# Autodesk Inventor assembly: HalfElevatpr
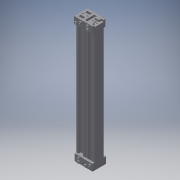
[picture p0: Inventor's stored thumbnail of the model, 180x180]
Saved by Autodesk Inventor 2019 (Build 230136000, 136)
## iProperties
Created: 2019-09-28
Part Number: HalfElevatpr
Document SubType Name: Assembly
Designer: james
Author: james
## Documents named in this file (5)
- F:\JimsDesign\Jims2020FTC\HalfElevatpr.iam
- F:\JimsDesign\Jims2020FTC\LeftSideElevator.ipt
- F:\JimsDesign\Library\McMaster\SocketScrews\91251A197_BLACK-OXIDE ALLOY STEEL SOCKET HEAD CAP SCREW.ipt
- F:\JimsDesign\Jims2020FTC\SliderLeft.iam
- F:\JimsDesign\Jims2020FTC\SliderRight.iam
## Components (8 placed, 4 different names)
1. LeftSideElevator:1 — Mate:8, Mate:9, Mate:14, Mate:15, Flush:2
2. LeftSideElevator:2 — Mate:16, Mate:17, Mate:18, Mate:19, Flush:3, Mate:20, Mate:21, Flush:4
3. 91251A197_BLACK-OXIDE ALLOY STEEL SOCKET HEAD CAP SCREW:1 — Mate:12, Mate:13
4. 91251A197_BLACK-OXIDE ALLOY STEEL SOCKET HEAD CAP SCREW:2 — Mate:8, Mate:11
5. SliderLeft:1 [sub-assembly] — Mate:9, Mate:11, Mate:12, Mate:13
6. SliderRight:1 [sub-assembly] — Mate:14, Mate:15, Flush:2, Mate:16, Mate:17
7. SliderLeft:2 [sub-assembly] — Mate:18, Mate:19, Flush:3
8. SliderRight:2 [sub-assembly] — Mate:20, Mate:21, Flush:4
## Relationships (16: Mate 13, Flush 3)
- Mate:8: LeftSideElevator:1 ↔ 91251A197_BLACK-OXIDE ALLOY STEEL SOCKET HEAD CAP SCREW:2
- Mate:9: LeftSideElevator:1 ↔ SliderLeft:1
- Mate:11: 91251A197_BLACK-OXIDE ALLOY STEEL SOCKET HEAD CAP SCREW:2 ↔ SliderLeft:1
- Mate:12: 91251A197_BLACK-OXIDE ALLOY STEEL SOCKET HEAD CAP SCREW:1 ↔ SliderLeft:1
- Mate:13: 91251A197_BLACK-OXIDE ALLOY STEEL SOCKET HEAD CAP SCREW:1 ↔ SliderLeft:1
- Mate:14: LeftSideElevator:1 ↔ SliderRight:1
- Mate:15: LeftSideElevator:1 ↔ SliderRight:1
- Flush:2: LeftSideElevator:1 ↔ SliderRight:1
- Mate:16: LeftSideElevator:2 ↔ SliderRight:1
- Mate:17: LeftSideElevator:2 ↔ SliderRight:1
- Mate:18: LeftSideElevator:2 ↔ SliderLeft:2
- Mate:19: LeftSideElevator:2 ↔ SliderLeft:2
- Flush:3: LeftSideElevator:2 ↔ SliderLeft:2
- Mate:20: LeftSideElevator:2 ↔ SliderRight:2
- Mate:21: LeftSideElevator:2 ↔ SliderRight:2
- Flush:4: LeftSideElevator:2 ↔ SliderRight:2
